# Autodesk Inventor assembly: car assembly Render
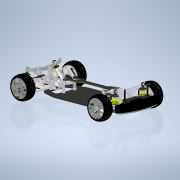
[picture p0: Inventor's stored thumbnail of the model, 180x180]
Saved by Autodesk Inventor 2020 (Build 240168000, 168)
## iProperties
Created: 2015-04-18
Part Number: car assembly Render
Document SubType Name: Assembly
Designer: Station9
Author: Station9
## Documents named in this file (12)
- C:\Users\0x6f736f646f\Documents\EurekaAutonomousCar\Src\Prototyping\Mechanical\chassis_ver1\car assembly Render.iam
- C:\Users\0x6f736f646f\Documents\EurekaAutonomousCar\Src\Prototyping\Mechanical\chassis_ver1\WSC2011_T05_M1_WHEEL.ipt
- C:\Users\0x6f736f646f\Documents\EurekaAutonomousCar\Src\Prototyping\Mechanical\chassis_ver1\WSC2011_TP05_01_CHASSIS.ipt
- C:\Users\0x6f736f646f\Documents\EurekaAutonomousCar\Src\Prototyping\Mechanical\chassis_ver1\WSC2011_TP05_01_FRONT.ipt
- C:\Users\0x6f736f646f\Documents\EurekaAutonomousCar\Src\Prototyping\Mechanical\chassis_ver1\LEFT REAR BUKHEAD.iam
- C:\Users\0x6f736f646f\Documents\EurekaAutonomousCar\Src\Prototyping\Mechanical\chassis_ver1\REAR RIGHT BUKHEAD.iam
- C:\Users\0x6f736f646f\Documents\EurekaAutonomousCar\Src\Prototyping\Mechanical\chassis_ver1\300-009 (TURNBUCKLE ASSEMBLY).iam
- C:\Users\0x6f736f646f\Documents\EurekaAutonomousCar\Src\Prototyping\Mechanical\chassis_ver1\300-031 (BODY SUPPORT).iam
- C:\Users\0x6f736f646f\Documents\EurekaAutonomousCar\Src\Prototyping\Mechanical\chassis_ver1\HUB ASSEMBLY.iam
- C:\Users\0x6f736f646f\Documents\EurekaAutonomousCar\Src\Prototyping\Mechanical\chassis_ver1\SUPPORT.iam
- C:\Users\0x6f736f646f\Documents\EurekaAutonomousCar\Src\Prototyping\Mechanical\chassis_ver1\SUSPENSION UNIT.iam
- E:\worldskills Project\Project Archive\AD\AD-6(94.01.29)WSC2011\1.ipt
## Components (18 placed, 11 different names)
1. WSC2011_TP05_01_CHASSIS:1 — Insert:1, Angle:1, Insert:2, Angle:2, Angle:4, Flush:1
2. WSC2011_TP05_01_FRONT:1 — Insert:3, Angle:3, Mate:6, Mate:7, Mate:8, Mate:9
3. LEFT REAR BUKHEAD:1 [sub-assembly] — Insert:2, Angle:2, Mate:2, Mate:12, Insert:5
4. REAR RIGHT BUKHEAD:1 [sub-assembly] — Insert:1, Angle:1, Insert:3, Angle:3, Mate:1, Mate:3, Mate:31
5. 300-009 (TURNBUCKLE ASSEMBLY):1 [sub-assembly] — Insert:4
6. 300-031 (BODY SUPPORT):1 [sub-assembly] — Insert:5
7. SUPPORT:1 [sub-assembly] — Mate:1, Mate:2, Mate:3, Mate:12, Mate:13, Mate:16, Mate:22, Mate:24, Insert:6, Mate:28, Mate:31, Mate:32, Mate:33
8. SUSPENSION UNIT:1 [sub-assembly] — Mate:13, Mate:22, Insert:6, Mate:28
9. 1:1
10. WSC2011_T05_M1_WHEEL:3 — Mate:8, Mate:9
11. WSC2011_T05_M1_WHEEL:4 — Mate:6, Mate:7
12. HUB ASSEMBLY:1 [sub-assembly] — Mate:16, Mate:24, Mate:26, Mate:27, Insert:4
13. WSC2011_T05_M1_WHEEL:5 — Mate:26, Mate:27, Angle:4
14. 300-009 (TURNBUCKLE ASSEMBLY):2 [sub-assembly] — Insert:7
15. 300-031 (BODY SUPPORT):2 [sub-assembly]
16. SUSPENSION UNIT:2 [sub-assembly]
17. HUB ASSEMBLY:2 [sub-assembly] — Insert:7, Mate:29, Mate:30, Mate:32, Mate:33
18. WSC2011_T05_M1_WHEEL:6 — Mate:29, Mate:30
## Relationships (32: Mate 20, Insert 7, Angle 4, Flush 1)
- Insert:1: WSC2011_TP05_01_CHASSIS:1 ↔ REAR RIGHT BUKHEAD:1
- Angle:1 (0 deg): WSC2011_TP05_01_CHASSIS:1 ↔ REAR RIGHT BUKHEAD:1
- Insert:2: WSC2011_TP05_01_CHASSIS:1 ↔ LEFT REAR BUKHEAD:1
- Angle:2 (0 deg): WSC2011_TP05_01_CHASSIS:1 ↔ LEFT REAR BUKHEAD:1
- Insert:3: WSC2011_TP05_01_FRONT:1 ↔ REAR RIGHT BUKHEAD:1
- Angle:3 (0 deg): WSC2011_TP05_01_FRONT:1 ↔ REAR RIGHT BUKHEAD:1
- Mate:1: REAR RIGHT BUKHEAD:1 ↔ SUPPORT:1
- Mate:2: LEFT REAR BUKHEAD:1 ↔ SUPPORT:1
- Mate:3: REAR RIGHT BUKHEAD:1 ↔ SUPPORT:1
- Mate:6: WSC2011_TP05_01_FRONT:1 ↔ WSC2011_T05_M1_WHEEL:4
- Mate:7: WSC2011_TP05_01_FRONT:1 ↔ WSC2011_T05_M1_WHEEL:4
- Mate:8: WSC2011_TP05_01_FRONT:1 ↔ WSC2011_T05_M1_WHEEL:3
- Mate:9: WSC2011_TP05_01_FRONT:1 ↔ WSC2011_T05_M1_WHEEL:3
- Mate:12: LEFT REAR BUKHEAD:1 ↔ SUPPORT:1
- Mate:13: SUPPORT:1 ↔ SUSPENSION UNIT:1
- Mate:16: SUPPORT:1 ↔ HUB ASSEMBLY:1
- Mate:22: SUPPORT:1 ↔ SUSPENSION UNIT:1
- Mate:24 (0.75 mm): SUPPORT:1 ↔ HUB ASSEMBLY:1
- Mate:26: HUB ASSEMBLY:1 ↔ WSC2011_T05_M1_WHEEL:5
- Mate:27: HUB ASSEMBLY:1 ↔ WSC2011_T05_M1_WHEEL:5
- Angle:4 (0 deg): WSC2011_TP05_01_CHASSIS:1 ↔ WSC2011_T05_M1_WHEEL:5
- Insert:4: 300-009 (TURNBUCKLE ASSEMBLY):1 ↔ HUB ASSEMBLY:1
- Insert:5: LEFT REAR BUKHEAD:1 ↔ 300-031 (BODY SUPPORT):1
- Insert:6: SUPPORT:1 ↔ SUSPENSION UNIT:1
- Mate:28 (4.028 mm): SUPPORT:1 ↔ SUSPENSION UNIT:1
- Flush:1 (-58 mm): WSC2011_TP05_01_CHASSIS:1
- Insert:7: 300-009 (TURNBUCKLE ASSEMBLY):2 ↔ HUB ASSEMBLY:2
- Mate:29: HUB ASSEMBLY:2 ↔ WSC2011_T05_M1_WHEEL:6
- Mate:30: HUB ASSEMBLY:2 ↔ WSC2011_T05_M1_WHEEL:6
- Mate:31: REAR RIGHT BUKHEAD:1 ↔ SUPPORT:1
- Mate:32: SUPPORT:1 ↔ HUB ASSEMBLY:2
- Mate:33 (0.75 mm): SUPPORT:1 ↔ HUB ASSEMBLY:2
